# Autodesk Inventor assembly: Assembly_Guinardia_V1
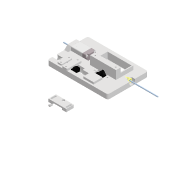
[picture p0: Inventor's stored thumbnail of the model, 180x180]
Saved by Autodesk Inventor 2022 (Build 260153000, 153)
## iProperties
Created: 2022-04-18
Part Number: Assembly_Guinardia_V1
Document SubType Name: Assembly
Designer: Prakash Lab
Author: Prakash Lab
## Documents named in this file (14)
- C:\Users\UC2\Documents\GitHub\Guinardia\INVENTOR\Assembly_Guinardia_V1.iam
- C:\Users\UC2\Documents\GitHub\Guinardia\INVENTOR\00_NEMA8.ipt
- C:\Users\UC2\Documents\GitHub\Guinardia\INVENTOR\00_CCTV_lens_M12_25mm_5mp.ipt
- C:\Users\UC2\Documents\GitHub\Guinardia\INVENTOR\00_coverslip_24x50mm.ipt
- C:\Users\UC2\Documents\GitHub\Guinardia\INVENTOR\00_PipetteTip200ul-1.ipt
- C:\Users\UC2\Documents\GitHub\Guinardia\INVENTOR\00_FEP_tube_2.2x0.5mm.ipt
- C:\Users\UC2\Documents\GitHub\Guinardia\INVENTOR\10_LED_cylnderlensmount.ipt
- C:\Users\UC2\Documents\GitHub\Guinardia\INVENTOR\10_Wellplate_base_v1.ipt
- C:\Users\UC2\Documents\GitHub\Guinardia\INVENTOR\00_HuaweiP30_Telelens_prismonly.ipt
- C:\Users\UC2\Documents\GitHub\Guinardia\INVENTOR\20_SMAConnector_fiber.ipt
- C:\Users\UC2\Documents\GitHub\Guinardia\INVENTOR\20_M12_Lens_Fixation_1.ipt
- C:\Users\UC2\Documents\GitHub\Guinardia\INVENTOR\20_Laserlauncher_Fixation.ipt
- C:\Users\UC2\Documents\GitHub\Guinardia\INVENTOR\20_Scanner_Fixation.ipt
- C:\Users\UC2\Documents\GitHub\Guinardia\INVENTOR\20_FEPTube_Motor_Clutch_1.ipt
## Components (16 placed, 13 different names)
1. 10_Wellplate_base_v1:1 — Mate:1, Mate:2, Mate:3, Mate:4, Mate:5, Flush:1, Mate:10, Flush:2, Mate:11, Mate:12, Einfügen:2, Winkel:1, Einfügen:3, Fluchtend:3, Fluchtend:4, Fluchtend:5, Fluchtend:6, Fluchtend:7, Fluchtend:8
2. 00_CCTV_lens_M12_25mm_5mp:1 — Mate:6, Flush:1, Passend:17, Passend:18
3. 00_coverslip_24x50mm:1 — Mate:1, Mate:2, Mate:3, Mate:7, Mate:13
4. 00_PipetteTip200ul-1:2 — Mate:9, Flush:2
5. 00_FEP_tube_2.2x0.5mm:1 — Mate:4, Mate:5, Mate:8, Mate:9, Mate:7
6. 00_PipetteTip200ul-1:3 — Mate:8, Mate:6, Mate:10
7. 00_coverslip_24x50mm:2 — Mate:11, Mate:12, Mate:13
8. 00_NEMA8:1 — Einfügen:2, Winkel:1
9. 00_HuaweiP30_Telelens_prismonly:1 — Passend:17, Passend:18
10. 10_LED_cylnderlensmount:1
11. 00_CCTV_lens_M12_25mm_5mp:2
12. 20_SMAConnector_fiber:1 — Einfügen:3
13. 20_M12_Lens_Fixation_1:1 — Fluchtend:3, Fluchtend:4
14. 20_Laserlauncher_Fixation:1 — Fluchtend:5, Fluchtend:6
15. 20_Scanner_Fixation:1 — Fluchtend:7, Fluchtend:8
16. 20_FEPTube_Motor_Clutch_1:1
## Relationships (26: Mate 15, Flush 8, Insert 2, Angle 1)
- Mate:1: 10_Wellplate_base_v1:1 ↔ 00_coverslip_24x50mm:1
- Mate:2: 10_Wellplate_base_v1:1 ↔ 00_coverslip_24x50mm:1
- Mate:3: 10_Wellplate_base_v1:1 ↔ 00_coverslip_24x50mm:1
- Mate:4 (-6 mm): 10_Wellplate_base_v1:1 ↔ 00_FEP_tube_2.2x0.5mm:1
- Mate:5: 10_Wellplate_base_v1:1 ↔ 00_FEP_tube_2.2x0.5mm:1
- Mate:8: 00_FEP_tube_2.2x0.5mm:1 ↔ 00_PipetteTip200ul-1:3
- Mate:9: 00_PipetteTip200ul-1:2 ↔ 00_FEP_tube_2.2x0.5mm:1
- Mate:6: 00_CCTV_lens_M12_25mm_5mp:1 ↔ 00_PipetteTip200ul-1:3
- Flush:1: 10_Wellplate_base_v1:1 ↔ 00_CCTV_lens_M12_25mm_5mp:1
- Mate:7 (3 mm): 00_coverslip_24x50mm:1 ↔ 00_FEP_tube_2.2x0.5mm:1
- Mate:10 (4 mm): 10_Wellplate_base_v1:1 ↔ 00_PipetteTip200ul-1:3
- Flush:2 (5 mm): 10_Wellplate_base_v1:1 ↔ 00_PipetteTip200ul-1:2
- Mate:11: 10_Wellplate_base_v1:1 ↔ 00_coverslip_24x50mm:2
- Mate:12: 10_Wellplate_base_v1:1 ↔ 00_coverslip_24x50mm:2
- Mate:13: 00_coverslip_24x50mm:1 ↔ 00_coverslip_24x50mm:2
- Einfügen:2 [Insert]: 10_Wellplate_base_v1:1 ↔ 00_NEMA8:1
- Winkel:1 [Angle] (0 deg): 10_Wellplate_base_v1:1 ↔ 00_NEMA8:1
- Passend:17 [Mate]: 00_CCTV_lens_M12_25mm_5mp:1 ↔ 00_HuaweiP30_Telelens_prismonly:1
- Passend:18 [Mate]: 00_CCTV_lens_M12_25mm_5mp:1 ↔ 00_HuaweiP30_Telelens_prismonly:1
- Einfügen:3 [Insert]: 10_Wellplate_base_v1:1 ↔ 20_SMAConnector_fiber:1
- Fluchtend:3 [Flush]: 10_Wellplate_base_v1:1 ↔ 20_M12_Lens_Fixation_1:1
- Fluchtend:4 [Flush]: 10_Wellplate_base_v1:1 ↔ 20_M12_Lens_Fixation_1:1
- Fluchtend:5 [Flush]: 10_Wellplate_base_v1:1 ↔ 20_Laserlauncher_Fixation:1
- Fluchtend:6 [Flush]: 10_Wellplate_base_v1:1 ↔ 20_Laserlauncher_Fixation:1
- Fluchtend:7 [Flush]: 10_Wellplate_base_v1:1 ↔ 20_Scanner_Fixation:1
- Fluchtend:8 [Flush]: 10_Wellplate_base_v1:1 ↔ 20_Scanner_Fixation:1
